# Autodesk Inventor assembly: Elevator Motor Assembly_MIR1 (nano)
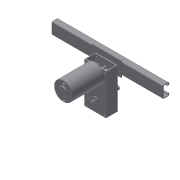
[picture p0: Inventor's stored thumbnail of the model, 180x180]
Saved by Autodesk Inventor 2015 (Build 190159000, 159)
## iProperties
Created: 2015-01-24
Part Number: Elevator Motor Assembly_MIR1 (nano)
Document SubType Name: Assembly
Designer: Peter
Author: Peter
## Documents named in this file (4)
- C:\Users\Noah\Desktop\FIRST-Team-1719-CAD-Team\2015 Robot CAD\Lifter Super Structure\Tower\Elevator Motor Assembly\Elevator Motor Assembly_MIR1 (nano).iam
- C:\Users\Noah\Desktop\FIRST-Team-1719-CAD-Team\2015 Robot CAD\Lifter Super Structure\Tower\Elevator Motor Assembly\Horizontal-Unistrut-Tower-Connector-15_MIR1.ipt
- C:\Users\Noah\Desktop\FIRST-Team-1719-CAD-Team\2015 Robot CAD\Lifter Super Structure\Tower\Elevator Motor Assembly\Andy Mark Tough Box Nano.iam
- C:\Users\Noah\Desktop\FIRST-Team-1719-CAD-Team\2015 Robot CAD\Lifter Super Structure\Tower\Elevator Motor Assembly\Nano Mounting Plate.ipt
## Components (3 placed, 3 different names)
1. Horizontal-Unistrut-Tower-Connector-15_MIR1:1 — Mate:2, Flush:1, Flush:2
2. Andy Mark Tough Box Nano:1 [sub-assembly] — Mate:1, Insert:1, Insert:2
3. Nano Mounting Plate:1 — Mate:1, Insert:1, Insert:2, Mate:2, Flush:1, Flush:2
## Relationships (6: Mate 2, Insert 2, Flush 2)
- Mate:1: Andy Mark Tough Box Nano:1 ↔ Nano Mounting Plate:1
- Insert:1: Andy Mark Tough Box Nano:1 ↔ Nano Mounting Plate:1
- Insert:2: Andy Mark Tough Box Nano:1 ↔ Nano Mounting Plate:1
- Mate:2: Horizontal-Unistrut-Tower-Connector-15_MIR1:1 ↔ Nano Mounting Plate:1
- Flush:1 (4.7625 mm): Horizontal-Unistrut-Tower-Connector-15_MIR1:1 ↔ Nano Mounting Plate:1
- Flush:2 (139.7 mm): Horizontal-Unistrut-Tower-Connector-15_MIR1:1 ↔ Nano Mounting Plate:1
